# Autodesk Inventor assembly: Eslabon interno
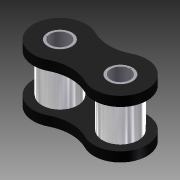
[picture p0: Inventor's stored thumbnail of the model, 180x180]
Saved by Autodesk Inventor 2011 (Build 150239000, 239)
## iProperties
Created: 2011-08-31
Part Number: Eslabon interno
Document SubType Name: Assembly
Designer: Luis
Author: Luis
## Documents named in this file (4)
- C:\Documents and Settings\Luis\Mis documentos\Inventor\Cadena 428\Eslabon interno.iam
- C:\Documents and Settings\Luis\Mis documentos\Inventor\Cadena 428\Concha2.ipt
- C:\Documents and Settings\Luis\Mis documentos\Inventor\Cadena 428\Buje.ipt
- C:\Documents and Settings\Luis\Mis documentos\Inventor\Cadena 428\Rodillo.ipt
## Components (6 placed, 3 different names)
1. Concha2:1 — Insert:1, Insert:2
2. Buje:1 — Insert:1, Insert:6
3. Buje:2 — Insert:2, Insert:5
4. Rodillo:1 — Insert:3
5. Rodillo:2 — Insert:4
6. Concha2:2 — Insert:3, Insert:4, Insert:5, Insert:6
## Relationships (6: Insert 6)
- Insert:1: Concha2:1 ↔ Buje:1
- Insert:2: Concha2:1 ↔ Buje:2
- Insert:3: Rodillo:1 ↔ Concha2:2
- Insert:4: Rodillo:2 ↔ Concha2:2
- Insert:5: Buje:2 ↔ Concha2:2
- Insert:6: Buje:1 ↔ Concha2:2
